# Autodesk Inventor assembly: ASY MSC 100 CONE
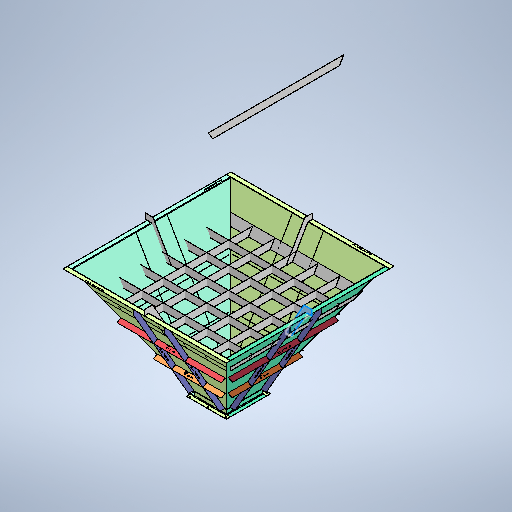
[picture p0: Inventor's stored thumbnail of the model, 512x512]
Saved by Autodesk Inventor 2025 (Build 290162010, 162A)
## iProperties
Created: 2024-05-19
Part Number: ASY MSC 100 CONE
Document SubType Name: Assembly
Designer: admin
Mass: 170206 g
Surface Area: 120081 cm^2
Volume: 21304.1 cm^3
Density: 7.98935 g/cm^3
Stock Number: ASY МОО 100 конус
Author: admin
## Documents named in this file (15)
- C:\Users\admin\YandexDisk-badmisterfox\домашниий пк\Inventor\NDM-VOS_powder_hopper\Workspaces\Workspace\Cone\ASY MSC 100 cone.iam
- C:\Users\admin\YandexDisk-badmisterfox\домашниий пк\Inventor\NDM-VOS_powder_hopper\Workspaces\Workspace\Cone\MSC 114 cone IN right board.ipt
- C:\Users\admin\YandexDisk-badmisterfox\домашниий пк\Inventor\NDM-VOS_powder_hopper\Workspaces\Workspace\Cone\MSC 113 cone IN left board.ipt
- C:\Users\admin\YandexDisk-badmisterfox\домашниий пк\Inventor\NDM-VOS_powder_hopper\Workspaces\Workspace\Cone\MSC 112 cone IN back.ipt
- C:\Users\admin\YandexDisk-badmisterfox\домашниий пк\Inventor\NDM-VOS_powder_hopper\Workspaces\Workspace\Cone\MSC DIM 001 cone sketch.ipt
- C:\Users\admin\YandexDisk-badmisterfox\домашниий пк\Inventor\NDM-VOS_powder_hopper\Workspaces\Workspace\Cone\MSC 115 cone IN bow.ipt
- C:\Users\admin\YandexDisk-badmisterfox\домашниий пк\Inventor\NDM-VOS_powder_hopper\Workspaces\Workspace\Cone\MSC 110 stringer cone.ipt
- C:\Users\admin\YandexDisk-badmisterfox\домашниий пк\Inventor\NDM-VOS_powder_hopper\Workspaces\Workspace\Cone\MSC 106 rib cone.ipt
- C:\Users\admin\YandexDisk-badmisterfox\домашниий пк\Inventor\NDM-VOS_powder_hopper\Workspaces\Workspace\Cone\MSC 107 rib cone.ipt
- C:\Users\admin\YandexDisk-badmisterfox\домашниий пк\Inventor\NDM-VOS_powder_hopper\Workspaces\Workspace\Cone\MSC 108 rib cone.ipt
- C:\Users\admin\YandexDisk-badmisterfox\домашниий пк\Inventor\NDM-VOS_powder_hopper\Workspaces\Workspace\Cone\MSC 109 rib cone.ipt
- C:\Users\admin\YandexDisk-badmisterfox\домашниий пк\Inventor\NDM-VOS_powder_hopper\NDM-VOS dummy2.ipt
- C:\Users\admin\YandexDisk-badmisterfox\домашниий пк\Inventor\NDM-VOS_powder_hopper\Workspaces\Workspace\Cone\MSC 201 GRID.ipt
- C:\Users\admin\YandexDisk-badmisterfox\домашниий пк\Inventor\NDM-VOS_powder_hopper\Workspaces\Workspace\Cone\MSC 202 GRID CORNER.ipt
- C:\Users\admin\YandexDisk-badmisterfox\домашниий пк\Inventor\NDM-VOS_powder_hopper\Workspaces\Workspace\Cone\MSC 206 GRID_CPY.ipt
## Components (42 placed, 20 different names)
1. NDM-VOS dummy2:1 — Mate:73, Mate:74, Flush:19
2. MSC DIM 001 CONE SKETCH:1 — Flush:8, Flush:9, Mate:1
3. MSC 112 CONE IN BACK:1 — Flush:6, Flush:10, Mate:2
4. MSC 114 CONE IN RIGHT BOARD:1 — Flush:13, Flush:15, Flush:18, Mate:79, Mate:81
5. MSC 113 CONE IN LEFT BOARD:1 — Mate:4, Flush:14, Mate:5
6. MSC 115 CONE IN BOW:1 — Mate:6, Flush:16, Flush:17, Mate:88
7. MSC 115 cone IN bow:2 — Mate:75, Flush:20, Flush:21, Mate:76, Mate:78, Mate:87
8. MSC 202 GRID CORNER:4
9. MSC 202 GRID CORNER:3
10. MSC 202 GRID CORNER:2 — Rigid:11
11. MSC 202 GRID CORNER:1 — Rigid:10
12. MSC 206 GRID_CPY:1 — Rigid:14
13. MSC 206 GRID_CPY:2 — Rigid:15, Mate:88
14. MSC 206 GRID_CPY:3 — Rigid:16
15. MSC 206 GRID_CPY:4 — Rigid:17
16. MSC 201 GRID:16 — Mate:87
17. MSC 106 RIB CONE:1 — Rigid:7, Rigid:8, Mate:77
18. MSC 109 RIB CONE:1 — Rigid:6
19. MSC 110 STRINGER CONE:4 — Rigid:4, Rigid:6, Mate:79, Mate:81
20. MSC 108 RIB CONE:1 — Rigid:4, Rigid:5, Mate:80
21. MSC 110 STRINGER CONE:3 — Rigid:5
22. MSC 110 STRINGER CONE:2 — Rigid:8, Rigid:9
23. MSC 107 RIB CONE:1 — Rigid:9
24. MSC 110 STRINGER CONE:1 — Rigid:7, Mate:76, Mate:78
25. MSC 106 rib cone:2
26. MSC 109 rib cone:2
27. MSC 110 stringer cone:6
28. MSC 108 rib cone:2
29. MSC 110 stringer cone:7
30. MSC 110 stringer cone:8
31. MSC 107 rib cone:2
32. MSC 110 stringer cone:9
33. MSC 201 GRID:2 — Mate:84, Mate:86, Rigid:15, Rigid:17, Flush:23
34. MSC 201 GRID:3
35. MSC 201 GRID:4
36. MSC 201 GRID:5
37. MSC 201 GRID:6
38. MSC 201 GRID:1 — Rigid:10, Rigid:11, Flush:22, Mate:83, Rigid:14, Rigid:16, Flush:23
39. MSC 201 GRID:10
40. MSC 201 GRID:11
41. MSC 201 GRID:12
42. MSC 201 GRID:13
## Component patterns: (2 elements, first: MSC 106 RIB CONE:1 + MSC 109 RIB CONE:1 + MSC 110 STRINGER CONE:4 + MSC 108 RIB CONE:1 + MSC 110 STRINGER CONE:3 + MSC 110 STRINGER CONE:2 + MSC 107 RIB CONE:1 + MSC 110 STRINGER CONE:1), (5 elements, first: MSC 201 GRID:2), (5 elements, first: MSC 201 GRID:1)
## Relationships (48: Mate 19, Flush 15, WeldJoint 14)
- Flush:6: MSC 112 CONE IN BACK:1
- Flush:8: MSC DIM 001 CONE SKETCH:1
- Flush:9: MSC DIM 001 CONE SKETCH:1
- Mate:1: MSC DIM 001 CONE SKETCH:1
- Flush:10: MSC 112 CONE IN BACK:1
- Mate:2: MSC 112 CONE IN BACK:1
- Flush:13: MSC 114 CONE IN RIGHT BOARD:1
- Mate:4: MSC 113 CONE IN LEFT BOARD:1
- Flush:14: MSC 113 CONE IN LEFT BOARD:1
- Mate:5: MSC 113 CONE IN LEFT BOARD:1
- Flush:15: MSC 114 CONE IN RIGHT BOARD:1
- Mate:6: MSC 115 CONE IN BOW:1
- Flush:16: MSC 115 CONE IN BOW:1
- Flush:17: MSC 115 CONE IN BOW:1
- Rigid:4 [WeldJoint] (2 mm): MSC 110 STRINGER CONE:4 ↔ MSC 108 RIB CONE:1
- Rigid:5 [WeldJoint] (2 mm): MSC 108 RIB CONE:1 ↔ MSC 110 STRINGER CONE:3
- Rigid:6 [WeldJoint] (2 mm): MSC 109 RIB CONE:1 ↔ MSC 110 STRINGER CONE:4
- Rigid:7 [WeldJoint] (2 mm): MSC 106 RIB CONE:1 ↔ MSC 110 STRINGER CONE:1
- Rigid:8 [WeldJoint] (2 mm): MSC 106 RIB CONE:1 ↔ MSC 110 STRINGER CONE:2
- Rigid:9 [WeldJoint] (2 mm): MSC 110 STRINGER CONE:2 ↔ MSC 107 RIB CONE:1
- Flush:18: MSC 114 CONE IN RIGHT BOARD:1
- Mate:73: NDM-VOS dummy2:1
- Mate:74: NDM-VOS dummy2:1
- Flush:19: NDM-VOS dummy2:1
- Mate:75: MSC 115 cone IN bow:2
- Flush:20: MSC 115 cone IN bow:2
- Flush:21: MSC 115 cone IN bow:2
- Mate:76: MSC 115 cone IN bow:2 ↔ MSC 110 STRINGER CONE:1
- Mate:77: MSC 106 RIB CONE:1
- Mate:78 (2 mm): MSC 115 cone IN bow:2 ↔ MSC 110 STRINGER CONE:1
- Mate:79: MSC 114 CONE IN RIGHT BOARD:1 ↔ MSC 110 STRINGER CONE:4
- Mate:80: MSC 108 RIB CONE:1
- Mate:81 (4 mm): MSC 114 CONE IN RIGHT BOARD:1 ↔ MSC 110 STRINGER CONE:4
- Rigid:10 [WeldJoint]: MSC 202 GRID CORNER:1 ↔ MSC 201 GRID:1
- Rigid:11 [WeldJoint]: MSC 202 GRID CORNER:2 ↔ MSC 201 GRID:1
- [WeldJoint]: MSC 202 GRID CORNER:3 ↔ MSC 201 GRID:2
- [WeldJoint]: MSC 202 GRID CORNER:4 ↔ MSC 201 GRID:2
- Flush:22: MSC 201 GRID:1
- Mate:83: MSC 201 GRID:1
- Mate:84: MSC 201 GRID:2
- Mate:86: MSC 201 GRID:2
- Rigid:14 [WeldJoint]: MSC 206 GRID_CPY:1 ↔ MSC 201 GRID:1
- Rigid:15 [WeldJoint]: MSC 206 GRID_CPY:2 ↔ MSC 201 GRID:2
- Rigid:16 [WeldJoint]: MSC 206 GRID_CPY:3 ↔ MSC 201 GRID:1
- Rigid:17 [WeldJoint]: MSC 206 GRID_CPY:4 ↔ MSC 201 GRID:2
- Mate:87: MSC 115 cone IN bow:2 ↔ MSC 201 GRID:16
- Flush:23: MSC 201 GRID:2 ↔ MSC 201 GRID:1
- Mate:88: MSC 115 CONE IN BOW:1 ↔ MSC 206 GRID_CPY:2
## Named parameters: Конус_Базовая_Высота = 1170 mm, Конус_отступ_от_пола = 0 mm, d200_d198 = 0 mm, d201_d199 = 0 mm
